# Autodesk Inventor assembly: pirxMainAssembly
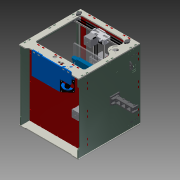
[picture p0: Inventor's stored thumbnail of the model, 180x180]
Saved by Autodesk Inventor 2013 (Build 170138000, 138)
## iProperties
Created: 2015-01-14
Part Number: pirxMainAssembly
Document SubType Name: Assembly
Designer: dzban
Author: dzban
## Documents named in this file (30)
- D:\PIRX\Artisan\OPENSOURCE\pirxMainAssembly.iam
- D:\PIRX\Artisan\OPENSOURCE\Case\caseTop.ipt
- D:\PIRX\Artisan\OPENSOURCE\Case\caseBack.ipt
- D:\PIRX\Artisan\OPENSOURCE\Case\caseBottom.ipt
- D:\PIRX\Artisan\OPENSOURCE\Case\caseFront.ipt
- D:\PIRX\Artisan\OPENSOURCE\Case\caseLeft.ipt
- D:\PIRX\Artisan\OPENSOURCE\Case\caseRight.ipt
- D:\PIRX\Artisan\OPENSOURCE\Case\boardCaseSide.ipt
- D:\PIRX\Artisan\OPENSOURCE\Case\boardCaseBack.ipt
- D:\PIRX\Artisan\OPENSOURCE\Case\boardCaseBottom.ipt
- D:\PIRX\Artisan\OPENSOURCE\XCars\Xcr.iam
- D:\PIRX\Artisan\OPENSOURCE\SmallPieces\spoolHolderHolder.ipt
- D:\PIRX\Artisan\OPENSOURCE\SmallPieces\spoolHolder.iam
- D:\PIRX\Artisan\OPENSOURCE\SmallPieces\bowdenHolder.ipt
- D:\PIRX\Artisan\OPENSOURCE\SmallPieces\xMotor.iam
- D:\PIRX\Artisan\OPENSOURCE\SmallPieces\xShaft.iam
- D:\PIRX\Artisan\OPENSOURCE\SmallPieces\xDriveShaftFront.iam
- D:\PIRX\Artisan\OPENSOURCE\SmallPieces\xDriveShaftBack.iam
- D:\PIRX\Artisan\OPENSOURCE\ZCar\Zshaft.ipt
- D:\PIRX\Artisan\OPENSOURCE\SmallPieces\shaftPlug22.ipt
- D:\PIRX\Artisan\OPENSOURCE\SmallPieces\shaftPlug24.ipt
- D:\PIRX\Artisan\OPENSOURCE\ZCar\zDrive.iam
- D:\PIRX\Artisan\OPENSOURCE\StockComponents\fan_60_60_10.ipt
- D:\PIRX\Artisan\OPENSOURCE\YCar\yCar.iam
- D:\PIRX\Artisan\OPENSOURCE\StockComponents\endstop.ipt
- D:\PIRX\Artisan\OPENSOURCE\StockComponents\endstopLever.ipt
- D:\PIRX\Artisan\OPENSOURCE\ZCar\zCar.iam
- D:\PIRX\Artisan\OPENSOURCE\StockComponents\printrboard.ipt
- D:\PIRX\Artisan\OPENSOURCE\StockComponents\gt2Belt188.ipt
- D:\PIRX\Artisan\OPENSOURCE\StockComponents\gt2Belt600.ipt
## Components (39 placed, 29 different names)
1. caseTop:1 — Mate:9, Mate:10, Mate:11, Angle:1, Angle:2, Insert:10, Insert:11, Insert:16, Insert:17, Insert:24, Insert:25, Angle:4, Angle:5
2. caseBack:1 — Mate:1, Mate:2, Flush:1, Mate:5, Mate:8, Mate:9, Mate:26, Mate:27, Tangent:1, Insert:5, Insert:6, Insert:7, Insert:8, Insert:30, Insert:31, Mate:35, Tangent:4, Tangent:5, Angle:3
3. caseBottom:1 — Mate:1, Mate:2, Flush:1, Mate:3, Mate:4, Mate:6, Mate:7, Mate:12, Mate:13, Mate:15, Mate:16, Mate:21, Insert:18, Insert:19, Insert:21, Insert:22, Insert:28, Insert:29, Insert:32, Insert:33
4. caseFront:1 — Mate:12, Mate:13, Mate:14
5. caseLeft:1 — Mate:6, Mate:7, Mate:8, Mate:10, Mate:11, Insert:12, Insert:13, Insert:14, Insert:15
6. caseRight:1 — Mate:3, Mate:4, Mate:5, Mate:14, Mate:17, Mate:18, Mate:19, Mate:20, Mate:22, Insert:3, Insert:4, Insert:9, Insert:20, Insert:23, Insert:26, Insert:27, Tangent:2, Mate:36, Tangent:6, Tangent:7
7. boardCaseSide:1 — Mate:15, Mate:16, Mate:21, Tangent:3, Flush:2, Mate:32
8. boardCaseBack:1 — Mate:17, Mate:18, Tangent:2
9. boardCaseBottom:1 — Mate:19, Mate:20, Mate:22
10. Xcr:1 [sub-assembly] — Mate:28, Angle:2, Mate:33, Mate:34, Mate:37, Mate:38
11. spoolHolderHolder:1 — Insert:30, Insert:31, Mate:29, Mate:30, Mate:31
12. spoolHolder:1 [sub-assembly] — Mate:29, Mate:30, Mate:31
13. bowdenHolder:1 — Mate:26, Mate:27, Tangent:1
14. xMotor:1 [sub-assembly] — Insert:9, Tangent:8
15. xShaft:1 [sub-assembly] — Insert:7, Insert:8, Mate:28
16. xShaft:2 [sub-assembly] — Insert:5, Insert:6
17. xDriveShaftFront:1 [sub-assembly] — Insert:4
18. xDriveShaftBack:1 [sub-assembly] — Insert:3, Angle:1, Insert:34, Insert:35, Insert:36
19. Zshaft:1 — Insert:10, Mate:39
20. Zshaft:2 — Insert:11
21. shaftPlug22:1 — Insert:19, Insert:21
22. shaftPlug22:2 — Insert:18, Insert:22
23. shaftPlug22:3 — Insert:17, Insert:24
24. shaftPlug22:4 — Insert:14, Insert:15
25. shaftPlug22:5 — Insert:16, Insert:25
26. shaftPlug22:6 — Insert:20, Insert:23
27. shaftPlug22:7 — Insert:12, Insert:13
28. shaftPlug24:1 — Insert:26, Insert:27
29. zDrive:1 [sub-assembly] — Insert:28, Insert:29
30. fan_60_60_10:1 — Tangent:3, Flush:2, Mate:32
31. yCar:1 [sub-assembly] — Mate:33, Mate:34
32. endstop:1 — Mate:35, Tangent:4, Tangent:5
33. endstopLever:1 — Mate:36, Tangent:6, Tangent:7
34. endstopLever:2 — Mate:37, Mate:38
35. zCar:1 [sub-assembly] — Mate:39, Angle:3
36. printrboard:1 — Insert:32, Insert:33
37. gt2Belt188:1 — Insert:34, Tangent:8
38. gt2Belt600:1 — Insert:36, Angle:5
39. gt2Belt600:2 — Insert:35, Angle:4
## Relationships (85: Mate 36, Insert 34, Tangent 8, Angle 5, Flush 2)
- Mate:1: caseBack:1 ↔ caseBottom:1
- Mate:2: caseBack:1 ↔ caseBottom:1
- Flush:1: caseBack:1 ↔ caseBottom:1
- Mate:3: caseBottom:1 ↔ caseRight:1
- Mate:4: caseBottom:1 ↔ caseRight:1
- Mate:5: caseBack:1 ↔ caseRight:1
- Mate:6: caseBottom:1 ↔ caseLeft:1
- Mate:7: caseBottom:1 ↔ caseLeft:1
- Mate:8: caseBack:1 ↔ caseLeft:1
- Mate:9: caseTop:1 ↔ caseBack:1
- Mate:10: caseTop:1 ↔ caseLeft:1
- Mate:11: caseTop:1 ↔ caseLeft:1
- Mate:12: caseBottom:1 ↔ caseFront:1
- Mate:13: caseBottom:1 ↔ caseFront:1
- Mate:14: caseFront:1 ↔ caseRight:1
- Mate:15: caseBottom:1 ↔ boardCaseSide:1
- Mate:16: caseBottom:1 ↔ boardCaseSide:1
- Mate:17: caseRight:1 ↔ boardCaseBack:1
- Mate:18: caseRight:1 ↔ boardCaseBack:1
- Mate:19: caseRight:1 ↔ boardCaseBottom:1
- Mate:20: caseRight:1 ↔ boardCaseBottom:1
- Mate:21: caseBottom:1 ↔ boardCaseSide:1
- Mate:22: caseRight:1 ↔ boardCaseBottom:1
- Mate:26: caseBack:1 ↔ bowdenHolder:1
- Mate:27: caseBack:1 ↔ bowdenHolder:1
- Tangent:1: caseBack:1 ↔ bowdenHolder:1
- Insert:3 (-5 mm): caseRight:1 ↔ xDriveShaftBack:1
- Insert:4 (-5 mm): caseRight:1 ↔ xDriveShaftFront:1
- Angle:1 (0 deg): caseTop:1 ↔ xDriveShaftBack:1
- Insert:5: caseBack:1 ↔ xShaft:2
- Insert:6: caseBack:1 ↔ xShaft:2
- Insert:7: caseBack:1 ↔ xShaft:1
- Insert:8: caseBack:1 ↔ xShaft:1
- Mate:28: Xcr:1 ↔ xShaft:1
- Angle:2 (0 deg): caseTop:1 ↔ Xcr:1
- Insert:9: caseRight:1 ↔ xMotor:1
- Insert:10 (-6 mm): caseTop:1 ↔ Zshaft:1
- Insert:11 (-6 mm): caseTop:1 ↔ Zshaft:2
- Insert:12: caseLeft:1 ↔ shaftPlug22:7
- Insert:13: caseLeft:1 ↔ shaftPlug22:7
- Insert:14: caseLeft:1 ↔ shaftPlug22:4
- Insert:15: caseLeft:1 ↔ shaftPlug22:4
- Insert:16: caseTop:1 ↔ shaftPlug22:5
- Insert:17: caseTop:1 ↔ shaftPlug22:3
- Insert:18: caseBottom:1 ↔ shaftPlug22:2
- Insert:19: caseBottom:1 ↔ shaftPlug22:1
- Insert:20: caseRight:1 ↔ shaftPlug22:6
- Insert:21: caseBottom:1 ↔ shaftPlug22:1
- Insert:22: caseBottom:1 ↔ shaftPlug22:2
- Insert:23: caseRight:1 ↔ shaftPlug22:6
- Insert:24: caseTop:1 ↔ shaftPlug22:3
- Insert:25: caseTop:1 ↔ shaftPlug22:5
- Insert:26: caseRight:1 ↔ shaftPlug24:1
- Insert:27: caseRight:1 ↔ shaftPlug24:1
- Insert:28: caseBottom:1 ↔ zDrive:1
- Insert:29: caseBottom:1 ↔ zDrive:1
- Insert:30: caseBack:1 ↔ spoolHolderHolder:1
- Insert:31: caseBack:1 ↔ spoolHolderHolder:1
- Mate:29: spoolHolderHolder:1 ↔ spoolHolder:1
- Mate:30: spoolHolderHolder:1 ↔ spoolHolder:1
- Mate:31: spoolHolderHolder:1 ↔ spoolHolder:1
- Tangent:2: caseRight:1 ↔ boardCaseBack:1
- Tangent:3: boardCaseSide:1 ↔ fan_60_60_10:1
- Flush:2 (-2 mm): boardCaseSide:1 ↔ fan_60_60_10:1
- Mate:32: boardCaseSide:1 ↔ fan_60_60_10:1
- Mate:33: Xcr:1 ↔ yCar:1
- Mate:34: Xcr:1 ↔ yCar:1
- Mate:35: caseBack:1 ↔ endstop:1
- Tangent:4: caseBack:1 ↔ endstop:1
- Tangent:5: caseBack:1 ↔ endstop:1
- Mate:36: caseRight:1 ↔ endstopLever:1
- Tangent:6: caseRight:1 ↔ endstopLever:1
- Tangent:7: caseRight:1 ↔ endstopLever:1
- Mate:37: Xcr:1 ↔ endstopLever:2
- Mate:38: Xcr:1 ↔ endstopLever:2
- Mate:39: Zshaft:1 ↔ zCar:1
- Angle:3 (0 deg): caseBack:1 ↔ zCar:1
- Insert:32 (3 mm): caseBottom:1 ↔ printrboard:1
- Insert:33 (3 mm): caseBottom:1 ↔ printrboard:1
- Insert:34: xDriveShaftBack:1 ↔ gt2Belt188:1
- Tangent:8: xMotor:1 ↔ gt2Belt188:1
- Insert:35: xDriveShaftBack:1 ↔ gt2Belt600:2
- Angle:4 (0 deg): caseTop:1 ↔ gt2Belt600:2
- Insert:36: xDriveShaftBack:1 ↔ gt2Belt600:1
- Angle:5 (0 deg): caseTop:1 ↔ gt2Belt600:1
